# Autodesk Inventor assembly: SensorBox
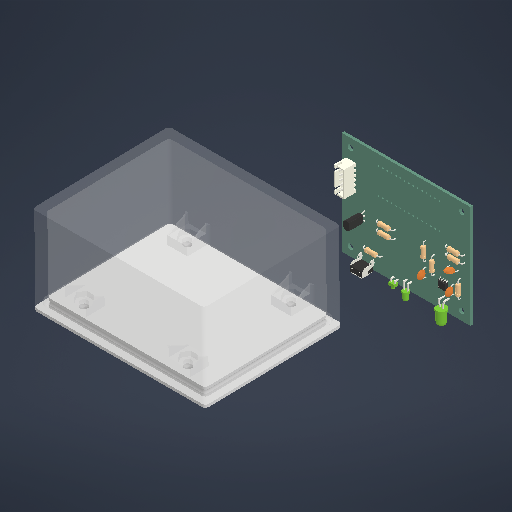
[picture p0: Inventor's stored thumbnail of the model, 512x512]
Saved by Autodesk Inventor 2026 (Build 300175000, 175)
## iProperties
Created: 2025-05-11
Part Number: SensorBox
Document SubType Name: Assembly
Designer: Riley
Author: Riley
## Documents named in this file (4)
- E:\IRGoKartTimingGate\CAD\SensorBox.iam
- E:\IRGoKartTimingGate\CAD\Amplifier\Amplifier\Amplifier.iam
- E:\IRGoKartTimingGate\CAD\Box.ipt
- E:\IRGoKartTimingGate\CAD\Lid.ipt
## Components (3 placed, 3 different names)
1. Amplifier:1 [sub-assembly]
2. Box:1 — Mate:1, Flush:1, Mate:2
3. Lid:1 — Mate:1, Flush:1, Mate:2
## Relationships (3: Mate 2, Flush 1)
- Mate:1: Box:1 ↔ Lid:1
- Flush:1: Box:1 ↔ Lid:1
- Mate:2: Box:1 ↔ Lid:1
